# Autodesk Inventor assembly: ABI_Baugruppe
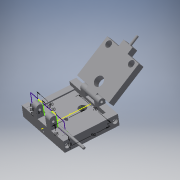
[picture p0: Inventor's stored thumbnail of the model, 180x180]
Saved by Autodesk Inventor 2018 (Build 220112000, 112)
## iProperties
Created: 2019-11-22
Part Number: ABI_Baugruppe
Material: Generisch
Document SubType Name: Assembly
Designer: Dubsky
Author: Dubsky
## Documents named in this file (9)
- C:\Users\Dubsky\Downloads\Biegevorrichtung\Daten\ABI_Baugruppe.iam
- C:\Users\Dubsky\Downloads\Biegevorrichtung\Daten\ABI_Arretierstift.ipt
- C:\Users\Dubsky\Downloads\Biegevorrichtung\Daten\ABI_Führungsblock.ipt
- C:\Users\Dubsky\Downloads\Biegevorrichtung\Daten\ABI_Grundplatte.ipt
- C:\Users\Dubsky\Downloads\Biegevorrichtung\Daten\ABI_Anschlag.ipt
- C:\Users\Dubsky\Downloads\Biegevorrichtung\Daten\ABI_Auswurf.ipt
- C:\Users\Dubsky\Downloads\Biegevorrichtung\Daten\ABI_Lagerbock.ipt
- C:\Users\Dubsky\Downloads\Biegevorrichtung\Daten\ABI_Stift.ipt
- C:\Users\Dubsky\Downloads\Biegevorrichtung\Daten\ABI_Deckel.ipt
## Components (8 placed, 8 different names)
1. ABI_Arretierstift:1 — Passend:31, Passend:32
2. ABI_Führungsblock:1 — Passend:10, Passend:11, Passend:12, Passend:13, Passend:26, Passend:27, Passend:31, Passend:32
3. ABI_Grundplatte:1 — Passend:24, Passend:25, Passend:26, Passend:27, Passend:28, Passend:29
4. ABI_Kasten:1 — Passend:10, Passend:13, Passend:14, Passend:15, Passend:29
5. ABI_Auswurf:1 — Passend:11, Passend:12, Passend:17, Passend:18
6. ABI_Lagerbock:1 — Passend:14, Passend:15, Passend:17, Passend:18, Passend:19, Passend:20, Passend:21, Passend:22, Passend:24, Passend:25, Passend:28
7. ABI_Stift:1 — Passend:23, Passend:30
8. ABI_Deckel:1 — Passend:19, Passend:20, Passend:21, Passend:22, Passend:23, Passend:30
## Relationships (22: Mate 22)
- Passend:10 [Mate]: ABI_Führungsblock:1 ↔ ABI_Kasten:1
- Passend:11 [Mate]: ABI_Führungsblock:1 ↔ ABI_Auswurf:1
- Passend:12 [Mate]: ABI_Führungsblock:1 ↔ ABI_Auswurf:1
- Passend:13 [Mate]: ABI_Führungsblock:1 ↔ ABI_Kasten:1
- Passend:14 [Mate]: ABI_Kasten:1 ↔ ABI_Lagerbock:1
- Passend:15 [Mate]: ABI_Kasten:1 ↔ ABI_Lagerbock:1
- Passend:17 [Mate]: ABI_Auswurf:1 ↔ ABI_Lagerbock:1
- Passend:18 [Mate]: ABI_Auswurf:1 ↔ ABI_Lagerbock:1
- Passend:19 [Mate]: ABI_Lagerbock:1 ↔ ABI_Deckel:1
- Passend:20 [Mate]: ABI_Lagerbock:1 ↔ ABI_Deckel:1
- Passend:21 [Mate]: ABI_Lagerbock:1 ↔ ABI_Deckel:1
- Passend:22 [Mate]: ABI_Lagerbock:1 ↔ ABI_Deckel:1
- Passend:23 [Mate]: ABI_Stift:1 ↔ ABI_Deckel:1
- Passend:24 [Mate]: ABI_Grundplatte:1 ↔ ABI_Lagerbock:1
- Passend:25 [Mate]: ABI_Grundplatte:1 ↔ ABI_Lagerbock:1
- Passend:26 [Mate]: ABI_Führungsblock:1 ↔ ABI_Grundplatte:1
- Passend:27 [Mate]: ABI_Führungsblock:1 ↔ ABI_Grundplatte:1
- Passend:28 [Mate]: ABI_Grundplatte:1 ↔ ABI_Lagerbock:1
- Passend:29 [Mate]: ABI_Grundplatte:1 ↔ ABI_Kasten:1
- Passend:30 [Mate]: ABI_Stift:1 ↔ ABI_Deckel:1
- Passend:31 [Mate]: ABI_Arretierstift:1 ↔ ABI_Führungsblock:1
- Passend:32 [Mate]: ABI_Arretierstift:1 ↔ ABI_Führungsblock:1
